# Autodesk Inventor assembly: Bearing Plate+Bearing
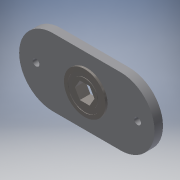
[picture p0: Inventor's stored thumbnail of the model, 180x180]
Saved by Autodesk Inventor 2019 (Build 230136000, 136)
## iProperties
Created: 2018-11-11
Part Number: Bearing Plate+Bearing
Document SubType Name: Assembly
Designer: maste
Author: maste
## Documents named in this file (3)
- D:\Summer Drive Base V1\Summer Drivebase\Bearing Plate+Bearing.iam
- D:\Summer Drive Base V1\Summer Drivebase\Bearing Plate.ipt
- D:\Summer Drive Base V1\Summer Drivebase\0_500_Hex_ID_x_1_125_OD_x_0_313_WD_Flanged_Bearing_v2_217-3875.ipt
## Components (2 placed, 2 different names)
1. Bearing Plate:1 — Mate:1, Mate:2
2. 0_500_Hex_ID_x_1_125_OD_x_0_313_WD_Flanged_Bearing_v2_217-3875:1 — Mate:1, Mate:2
## Relationships (2: Mate 2)
- Mate:1: Bearing Plate:1 ↔ 0_500_Hex_ID_x_1_125_OD_x_0_313_WD_Flanged_Bearing_v2_217-3875:1
- Mate:2: Bearing Plate:1 ↔ 0_500_Hex_ID_x_1_125_OD_x_0_313_WD_Flanged_Bearing_v2_217-3875:1
